# Autodesk Inventor assembly: Leg V3
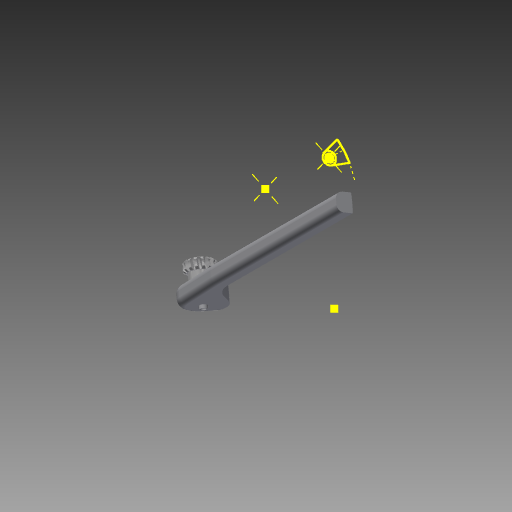
[picture p0: Inventor's stored thumbnail of the model, 512x512]
Saved by Autodesk Inventor 2019.1 (Build 231200000, 200)
## iProperties
Created: 2018-11-20
Part Number: Leg V3
Material: Generisch
Document SubType Name: Assembly
Designer: JochenAlt
Author: JochenAlt
## Documents named in this file (3)
- D:\Projects\Ondine\CAD\Leg\Leg V3.iam
- D:\Projects\Ondine\CAD\Leg\Leg V3.ipt
- D:\Projects\Ondine\CAD\Leg\Schnecke\Schneckenrad1.ipt
## Components (2 placed, 2 different names)
1. Leg V3:1 — Passend:1, Winkel:1, Passend:2
2. Schneckenrad:1 — Passend:1, Winkel:1, Passend:2
## Relationships (3: Mate 2, Angle 1)
- Passend:1 [Mate]: Leg V3:1 ↔ Schneckenrad:1
- Winkel:1 [Angle] (180 deg): Leg V3:1 ↔ Schneckenrad:1
- Passend:2 [Mate]: Leg V3:1 ↔ Schneckenrad:1
